# Autodesk Inventor assembly: rat_cap_walls_v8
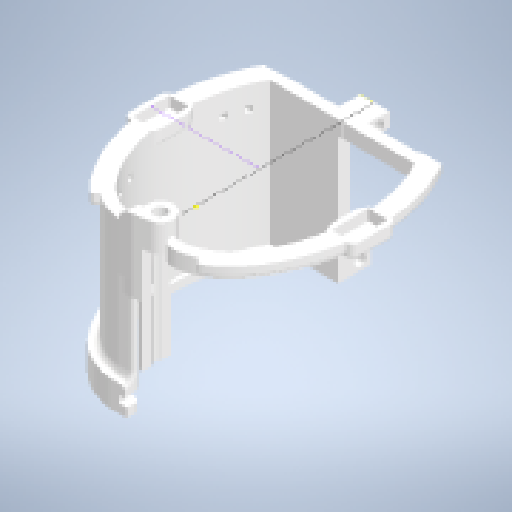
[picture p0: Inventor's stored thumbnail of the model, 512x512]
Saved by Autodesk Inventor 2025.2 (Build 292293000, 293)
## iProperties
Created: 2025-11-03
Part Number: rat_cap_walls_v8
Document SubType Name: Assembly
Designer: AdminForWorker
Title: rat_cap_walls_v8
Author: AdminForWorker
## Documents named in this file (3)
- C:\Users\AkramiLab\Downloads\rat_cap_EC_v12 v0\rat_cap_walls_v8.iam
- C:\Users\AkramiLab\Downloads\rat_cap_EC_v12 v0\rat_cap_left_wall_v8.ipt
- C:\Users\AkramiLab\Downloads\rat_cap_EC_v12 v0\rat_cap_right_wall_v8.ipt
## Components (2 placed, 2 different names)
1. rat_cap_left_wall_v8:1
2. rat_cap_right_wall_v8:1
## Named parameters: OuterWidth = 3 mm, OuterLength = 5.5 mm, InnerWidth = 1 mm, InnerLength = 5 mm
